# Autodesk Inventor assembly: RearAxle
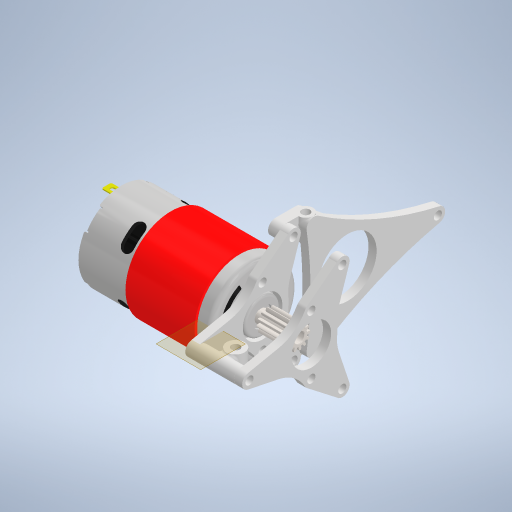
[picture p0: Inventor's stored thumbnail of the model, 512x512]
Saved by Autodesk Inventor 2024 (Build 280153020, 153B)
## iProperties
Created: 2024-04-17
Part Number: RearAxle
Document SubType Name: Assembly
Designer: lvrectanus0
Author: lvrectanus0
## Documents named in this file (5)
- C:\Users\lvrectanus0\Documents\Github\SPARKLabs-ArduinoProjects\project\CAD\RearAxle.iam
- C:\Users\lvrectanus0\Documents\Github\SPARKLabs-ArduinoProjects\project\CAD\am-3775a_12T 775 RedLine with 12T Pinion.iam
- C:\Users\lvrectanus0\Documents\Github\SPARKLabs-ArduinoProjects\project\CAD\MotorHolder.ipt
- C:\Users\lvrectanus0\Documents\Github\SPARKLabs-ArduinoProjects\project\CAD\AxleMount.ipt
- C:\Users\lvrectanus0\Documents\Github\SPARKLabs-ArduinoProjects\project\CAD\MotorMountSpacerConnector.ipt
## Components (5 placed, 4 different names)
1. am-3775a_12T 775 RedLine with 12T Pinion:1 [sub-assembly] — Flush:1
2. MotorHolder:1 — Flush:1, Flush:3, Flush:4, Mate:2
3. AxleMount:1 — Flush:3
4. MotorMountSpacerConnector:1 — Flush:4, Mate:1, Mate:3
5. MotorHolder:2 — Mate:1, Mate:2, Mate:3
## Relationships (6: Flush 3, Mate 3)
- Flush:1: am-3775a_12T 775 RedLine with 12T Pinion:1 ↔ MotorHolder:1
- Flush:3: MotorHolder:1 ↔ AxleMount:1
- Flush:4: MotorHolder:1 ↔ MotorMountSpacerConnector:1
- Mate:1: MotorMountSpacerConnector:1 ↔ MotorHolder:2
- Mate:2: MotorHolder:1 ↔ MotorHolder:2
- Mate:3: MotorMountSpacerConnector:1 ↔ MotorHolder:2
